# Autodesk Inventor assembly: vp6242
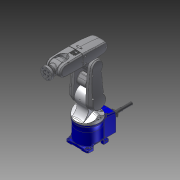
[picture p0: Inventor's stored thumbnail of the model, 180x180]
Saved by Autodesk Inventor 2013 (Build 170138000, 138)
## iProperties
Created: 2013-01-29
Part Number: vp6242
Document SubType Name: Assembly
Designer: Mahisorn
Author: Mahisorn
## Documents named in this file (10)
- E:\mahisorn\documents\hg-ros-pkg\cad\gripper\vp6242.iam
- E:\mahisorn\documents\hg-ros-pkg\cad\gripper\Imported Components\410590-0170-c001_drx\410590-0170-c001_drx.ipt
- E:\mahisorn\documents\hg-ros-pkg\cad\gripper\Imported Components\410590-0170-c002_drx\410590-0170-c002_drx.ipt
- E:\mahisorn\documents\hg-ros-pkg\cad\gripper\Imported Components\410590-0170-c003_drx\410590-0170-c003_drx.ipt
- E:\mahisorn\documents\hg-ros-pkg\cad\gripper\Imported Components\410590-0170-c004_drx\410590-0170-c004_drx.ipt
- E:\mahisorn\documents\hg-ros-pkg\cad\gripper\Imported Components\410590-0170-c005_drx\410590-0170-c005_drx.ipt
- E:\mahisorn\documents\hg-ros-pkg\cad\gripper\Imported Components\410590-0170-c006_drx\410590-0170-c006_drx.ipt
- E:\mahisorn\documents\hg-ros-pkg\cad\gripper\Plate.ipt
- E:\mahisorn\documents\Inventor\Content Center Files\R2013\en-US\ANSI B18.3.1M(3)\ANSI B18.3.1M - M5x0.8 x 12(5).ipt
- E:\mahisorn\documents\Inventor\Content Center Files\R2013\en-US\IFI 502(20)\IFI 502 - M6x1 x 20(2) T.ipt
## Components (15 placed, 9 different names)
1. Plate:1 — Mate:1, Insert:6, Insert:7, Insert:8, Insert:9, Insert:10, Insert:11, Insert:12, Insert:13
2. Drilled Broached Hexagon Socket Head Cap Screw - 6 Holes - Metric M5x0.8 x 12:2 — Insert:7
3. Drilled Broached Hexagon Socket Head Cap Screw - 6 Holes - Metric M5x0.8 x 12:3 — Insert:6
4. Drilled Broached Hexagon Socket Head Cap Screw - 6 Holes - Metric M5x0.8 x 12:4 — Insert:9
5. Drilled Broached Hexagon Socket Head Cap Screw - 6 Holes - Metric M5x0.8 x 12:5 — Insert:8
6. Fully Upset Hex Head Tapping Screw - Type T - Metric M6x1 x 20:1 — Insert:10
7. Fully Upset Hex Head Tapping Screw - Type T - Metric M6x1 x 20:2 — Insert:11
8. Fully Upset Hex Head Tapping Screw - Type T - Metric M6x1 x 20:4 — Insert:12
9. Fully Upset Hex Head Tapping Screw - Type T - Metric M6x1 x 20:5 — Insert:13
10. 410590-0170-c001_drx:1 — Insert:1
11. 410590-0170-c002_drx:1 — Insert:1, Insert:2
12. 410590-0170-c003_drx:1 — Insert:2, Insert:3
13. 410590-0170-c004_drx:1 — Insert:3, Insert:4
14. 410590-0170-c005_drx:1 — Insert:4, Insert:5
15. 410590-0170-c006_drx:1 — Insert:5, Mate:1
## Relationships (14: Insert 13, Mate 1)
- Insert:1: 410590-0170-c001_drx:1 ↔ 410590-0170-c002_drx:1
- Insert:2: 410590-0170-c002_drx:1 ↔ 410590-0170-c003_drx:1
- Insert:3: 410590-0170-c003_drx:1 ↔ 410590-0170-c004_drx:1
- Insert:4: 410590-0170-c004_drx:1 ↔ 410590-0170-c005_drx:1
- Insert:5: 410590-0170-c005_drx:1 ↔ 410590-0170-c006_drx:1
- Mate:1: Plate:1 ↔ 410590-0170-c006_drx:1
- Insert:6: Plate:1 ↔ Drilled Broached Hexagon Socket Head Cap Screw - 6 Holes - Metric M5x0.8 x 12:3
- Insert:7: Plate:1 ↔ Drilled Broached Hexagon Socket Head Cap Screw - 6 Holes - Metric M5x0.8 x 12:2
- Insert:8: Plate:1 ↔ Drilled Broached Hexagon Socket Head Cap Screw - 6 Holes - Metric M5x0.8 x 12:5
- Insert:9: Plate:1 ↔ Drilled Broached Hexagon Socket Head Cap Screw - 6 Holes - Metric M5x0.8 x 12:4
- Insert:10: Plate:1 ↔ Fully Upset Hex Head Tapping Screw - Type T - Metric M6x1 x 20:1
- Insert:11: Plate:1 ↔ Fully Upset Hex Head Tapping Screw - Type T - Metric M6x1 x 20:2
- Insert:12: Plate:1 ↔ Fully Upset Hex Head Tapping Screw - Type T - Metric M6x1 x 20:4
- Insert:13: Plate:1 ↔ Fully Upset Hex Head Tapping Screw - Type T - Metric M6x1 x 20:5
